# Autodesk Inventor assembly: module assembly
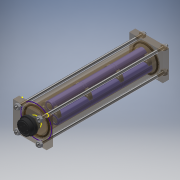
[picture p0: Inventor's stored thumbnail of the model, 180x180]
Saved by Autodesk Inventor 2017 (Build 210142000, 142)
## iProperties
Created: 2017-08-10
Part Number: module assembly
Document SubType Name: Assembly
Designer: Kai
Author: Kai
## Documents named in this file (11)
- C:\Users\Kai\Documents\Sub_stuff\2018sub\box2.0.1\assem\module assembly.iam
- C:\Users\Kai\Documents\Sub_stuff\2018sub\battery\18650.ipt
- C:\Users\Kai\Documents\Sub_stuff\2018sub\battery\battery_holder.ipt
- C:\Users\Kai\Documents\Sub_stuff\2018sub\battery\polycarb_back.ipt
- C:\Users\Kai\Documents\Sub_stuff\2018sub\battery\gasket.ipt
- C:\Users\Kai\Documents\Sub_stuff\2018sub\battery\tube.ipt
- C:\Users\Kai\Documents\Sub_stuff\2018sub\battery\polycarb_front.ipt
- C:\Users\Kai\Documents\Sub_stuff\2018sub\battery\rod.ipt
- C:\Users\Kai\Documents\Sub_stuff\2018sub\box2.0.1\assem\connector.ipt
- C:\Users\Kai\Documents\Sub_stuff\2018sub\battery\connector_nut.ipt
- C:\Users\Kai\Documents\Sub_stuff\2018sub\battery\6mm_nut.ipt
## Components (32 placed, 10 different names)
1. 18650:1 — Mate:7, Mate:8, Mate:9, Mate:10, Mate:18
2. 18650:2 — Mate:8, Mate:9, Mate:14
3. 18650:3 — Mate:1, Mate:4, Mate:15, Flush:5
4. 18650:4 — Mate:7, Mate:10, Flush:3, Mate:16
5. 18650:5 — Mate:5, Mate:6, Mate:11, Mate:12
6. 18650:6 — Mate:1, Mate:2, Mate:3, Mate:4, Mate:19, Mate:21
7. 18650:7 — Mate:2, Mate:3, Flush:1, Mate:17
8. 18650:8 — Mate:6, Mate:11, Mate:13, Flush:4, Mate:22
9. 18650:9 — Mate:5, Mate:12, Flush:2
10. battery_holder:1 — Mate:13, Mate:14, Mate:15, Flush:1, Flush:2, Flush:3, Mate:20
11. battery_holder:2 — Mate:16, Mate:17, Flush:4, Mate:24
12. battery_holder:3 — Mate:18, Mate:19, Mate:20, Mate:23
13. battery_holder:4 — Mate:21, Mate:22, Mate:23
14. polycarb_back:1 — Mate:27, Mate:28, Mate:29, Mate:58, Tangent:2, Mate:63, Flush:6, Mate:75, Mate:76, Mate:77, Mate:78
15. gasket:1 — Mate:26, Tangent:1
16. gasket:2 — Mate:25, Tangent:2
17. tube:1 — Mate:24, Flush:5, Mate:25, Mate:26, Mate:27, Mate:28, Mate:29, Mate:30, Mate:31, Mate:32
18. polycarb_front:1 — Mate:30, Mate:31, Mate:32, Mate:58, Tangent:1, Mate:59, Mate:60, Mate:61, Mate:64, Mate:65, Mate:66, Flush:7, Flush:8, Flush:9, Mate:67, Mate:68, Mate:69, Mate:70
19. connector:1 — Mate:59, Mate:60, Mate:62
20. connector_nut:1 — Mate:61, Mate:62
21. rod:1 — Mate:64, Flush:9, Mate:72, Mate:79
22. rod:2 — Mate:65, Flush:7, Mate:74, Mate:81
23. rod:3 — Mate:63, Flush:6, Mate:73, Mate:80
24. rod:4 — Mate:66, Flush:8, Mate:71, Mate:82
25. 6mm_nut:1 — Mate:68, Mate:71
26. 6mm_nut:2 — Mate:67, Mate:74
27. 6mm_nut:3 — Mate:70, Mate:72
28. 6mm_nut:4 — Mate:69, Mate:73
29. 6mm_nut:5 — Mate:75, Mate:82
30. 6mm_nut:6 — Mate:76, Mate:81
31. 6mm_nut:7 — Mate:77, Mate:80
32. 6mm_nut:8 — Mate:78, Mate:79
## Relationships (68: Mate 57, Flush 9, Tangent 2)
- Mate:1: 18650:3 ↔ 18650:6
- Mate:2: 18650:6 ↔ 18650:7
- Mate:3: 18650:6 ↔ 18650:7
- Mate:4: 18650:3 ↔ 18650:6
- Mate:5: 18650:5 ↔ 18650:9
- Mate:6: 18650:5 ↔ 18650:8
- Mate:7: 18650:1 ↔ 18650:4
- Mate:8: 18650:1 ↔ 18650:2
- Mate:9: 18650:1 ↔ 18650:2
- Mate:10: 18650:1 ↔ 18650:4
- Mate:11: 18650:5 ↔ 18650:8
- Mate:12: 18650:5 ↔ 18650:9
- Mate:13: 18650:8 ↔ battery_holder:1
- Mate:14: 18650:2 ↔ battery_holder:1
- Mate:15: 18650:3 ↔ battery_holder:1
- Flush:1: 18650:7 ↔ battery_holder:1
- Flush:2: 18650:9 ↔ battery_holder:1
- Flush:3: 18650:4 ↔ battery_holder:1
- Mate:16: 18650:4 ↔ battery_holder:2
- Mate:17: 18650:7 ↔ battery_holder:2
- Flush:4: 18650:8 ↔ battery_holder:2
- Mate:18: 18650:1 ↔ battery_holder:3
- Mate:19: 18650:6 ↔ battery_holder:3
- Mate:20 (58.42 mm): battery_holder:1 ↔ battery_holder:3
- Mate:21: 18650:6 ↔ battery_holder:4
- Mate:22: 18650:8 ↔ battery_holder:4
- Mate:23 (58.42 mm): battery_holder:3 ↔ battery_holder:4
- Mate:24: battery_holder:2 ↔ tube:1
- Flush:5 (6.35 mm): 18650:3 ↔ tube:1
- Mate:25: gasket:2 ↔ tube:1
- Mate:26: gasket:1 ↔ tube:1
- Mate:27: polycarb_back:1 ↔ tube:1
- Mate:28 (-28.575 mm): polycarb_back:1 ↔ tube:1
- Mate:29 (-28.575 mm): polycarb_back:1 ↔ tube:1
- Mate:30: tube:1 ↔ polycarb_front:1
- Mate:31 (-28.575 mm): tube:1 ↔ polycarb_front:1
- Mate:32 (-28.575 mm): tube:1 ↔ polycarb_front:1
- Mate:58 (228.6 mm): polycarb_back:1 ↔ polycarb_front:1
- Tangent:1: gasket:1 ↔ polycarb_front:1
- Tangent:2: polycarb_back:1 ↔ gasket:2
- Mate:59: polycarb_front:1 ↔ connector:1
- Mate:60: polycarb_front:1 ↔ connector:1
- Mate:61: polycarb_front:1 ↔ connector_nut:1
- Mate:62: connector:1 ↔ connector_nut:1
- Mate:63: polycarb_back:1 ↔ rod:3
- Flush:6 (-7.62 mm): polycarb_back:1 ↔ rod:3
- Mate:64: polycarb_front:1 ↔ rod:1
- Mate:65: polycarb_front:1 ↔ rod:2
- Mate:66: polycarb_front:1 ↔ rod:4
- Flush:7 (-7.62 mm): polycarb_front:1 ↔ rod:2
- Flush:8 (-7.62 mm): polycarb_front:1 ↔ rod:4
- Flush:9 (-7.62 mm): polycarb_front:1 ↔ rod:1
- Mate:67: polycarb_front:1 ↔ 6mm_nut:2
- Mate:68: polycarb_front:1 ↔ 6mm_nut:1
- Mate:69: polycarb_front:1 ↔ 6mm_nut:4
- Mate:70: polycarb_front:1 ↔ 6mm_nut:3
- Mate:71: rod:4 ↔ 6mm_nut:1
- Mate:72: rod:1 ↔ 6mm_nut:3
- Mate:73: rod:3 ↔ 6mm_nut:4
- Mate:74: rod:2 ↔ 6mm_nut:2
- Mate:75: polycarb_back:1 ↔ 6mm_nut:5
- Mate:76: polycarb_back:1 ↔ 6mm_nut:6
- Mate:77: polycarb_back:1 ↔ 6mm_nut:7
- Mate:78: polycarb_back:1 ↔ 6mm_nut:8
- Mate:79: rod:1 ↔ 6mm_nut:8
- Mate:80: rod:3 ↔ 6mm_nut:7
- Mate:81: rod:2 ↔ 6mm_nut:6
- Mate:82: rod:4 ↔ 6mm_nut:5
